# Autodesk Inventor assembly: ARM_039_MiddleRoller
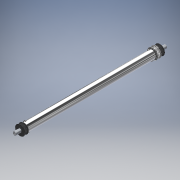
[picture p0: Inventor's stored thumbnail of the model, 180x180]
Saved by Autodesk Inventor 2018.3 (Build 223284000, 284)
## iProperties
Created: 2020-02-08
Part Number: ARM_039_MiddleRoller
Document SubType Name: Assembly
Designer: 22turnmaxw
Author: 22turnmaxw
## Documents named in this file (9)
- C:\Users\22barlalex\Documents\GrabCAD\Infinite Recharge 2020\Build season\ARM_039_MiddleRoller.iam
- C:\Users\22barlalex\Documents\GrabCAD\Infinite Recharge 2020\Build season\ARM_038_MiddleRollerTube.ipt
- C:\Users\22barlalex\Documents\GrabCAD\Infinite Recharge 2020\Build season\ARM_015_VersaRoller_Hub_1_2_Hex_Bore_x_1-1_8_OD_Aluminum_217-5895.ipt
- C:\Users\22barlalex\Documents\GrabCAD\Infinite Recharge 2020\Build season\ARM_034_36Tx9mm3mmPitchPulley.ipt
- C:\Users\22barlalex\Documents\GrabCAD\Infinite Recharge 2020\Build season\ARM_028_ANSI B18.3 - 10-24 UNC - UNC - 0.1875.ipt
- C:\Users\22barlalex\Documents\GrabCAD\Infinite Recharge 2020\Build season\ARM_027_ANSI B18.3 - 5_16-18 UNC - UNC - 0.5.ipt
- C:\Users\22barlalex\Documents\GrabCAD\Infinite Recharge 2020\Build season\ARM_044_SDP_a_6a53-040df0908.ipt
- C:\Users\22barlalex\Documents\GrabCAD\Infinite Recharge 2020\Build season\ARM_017_VersaRoller_1_2_Hex_Hub_Insert_1_2_Hex_Shaft_x_2-1_2_Long_217-5899.ipt
- C:\Users\22barlalex\Documents\GrabCAD\Infinite Recharge 2020\Build season\ARM_056_ActualMiddleRollerRightHexInsert.ipt
## Components (14 placed, 8 different names)
1. ARM_038_MiddleRollerTube:1 — Mate:1, Mate:2, Mate:3, Mate:4, Mate:32, Mate:33, Tangent:1, Mate:34, Tangent:2, Mate:35, Tangent:3, Mate:36, Tangent:4, Mate:72, Mate:91
2. ARM_015_VersaRoller_Hub_1_2_Hex_Bore_x_1-1_8_OD_Aluminum_217-5895:1 — Mate:1, Mate:2, Mate:32, Mate:80, Mate:90
3. ARM_015_VersaRoller_Hub_1_2_Hex_Bore_x_1-1_8_OD_Aluminum_217-5895:2 — Mate:3, Mate:4, Flush:1, Mate:88
4. ARM_034_36Tx9mm3mmPitchPulley:3 — Mate:70, Mate:71, Flush:1, Mate:87, Mate:89
5. Hexagon Socket Button Head Cap Screw - Inch 10 - 24 x 3/16:1 — Mate:33, Tangent:1
6. Hexagon Socket Button Head Cap Screw - Inch 10 - 24 x 3/16:2 — Mate:34, Tangent:2
7. Hexagon Socket Button Head Cap Screw - Inch 10 - 24 x 3/16:3 — Mate:35, Tangent:3
8. Hexagon Socket Button Head Cap Screw - Inch 10 - 24 x 3/16:4 — Mate:36, Tangent:4
9. Hexagon Socket Button Head Cap Screw - Inch 5/16 - 18 x 1/2:2
10. Hexagon Socket Button Head Cap Screw - Inch 5/16 - 18 x 1/2:3 — Mate:85, Mate:86, Mate:87
11. ARM_044_SDP_a_6a53-040df0908:1 — Mate:70, Mate:71, Mate:72, Mate:93
12. ARM_034_36Tx9mm3mmPitchPulley:4 — Mate:80, Mate:92
13. ARM_017_VersaRoller_1_2_Hex_Hub_Insert_1_2_Hex_Shaft_x_2-1_2_Long_217-5899:1 — Mate:85, Mate:86, Mate:88, Mate:89, Mate:93
14. ARM_056_ActualMiddleRollerRightHexInsert:1 — Mate:90, Mate:91, Mate:92
## Relationships (27: Mate 22, Tangent 4, Flush 1)
- Mate:1: ARM_038_MiddleRollerTube:1 ↔ ARM_015_VersaRoller_Hub_1_2_Hex_Bore_x_1-1_8_OD_Aluminum_217-5895:1
- Mate:2: ARM_038_MiddleRollerTube:1 ↔ ARM_015_VersaRoller_Hub_1_2_Hex_Bore_x_1-1_8_OD_Aluminum_217-5895:1
- Mate:3: ARM_038_MiddleRollerTube:1 ↔ ARM_015_VersaRoller_Hub_1_2_Hex_Bore_x_1-1_8_OD_Aluminum_217-5895:2
- Mate:4: ARM_038_MiddleRollerTube:1 ↔ ARM_015_VersaRoller_Hub_1_2_Hex_Bore_x_1-1_8_OD_Aluminum_217-5895:2
- Mate:32: ARM_038_MiddleRollerTube:1 ↔ ARM_015_VersaRoller_Hub_1_2_Hex_Bore_x_1-1_8_OD_Aluminum_217-5895:1
- Mate:33: ARM_038_MiddleRollerTube:1 ↔ Hexagon Socket Button Head Cap Screw - Inch 10 - 24 x 3/16:1
- Tangent:1: ARM_038_MiddleRollerTube:1 ↔ Hexagon Socket Button Head Cap Screw - Inch 10 - 24 x 3/16:1
- Mate:34: ARM_038_MiddleRollerTube:1 ↔ Hexagon Socket Button Head Cap Screw - Inch 10 - 24 x 3/16:2
- Tangent:2: ARM_038_MiddleRollerTube:1 ↔ Hexagon Socket Button Head Cap Screw - Inch 10 - 24 x 3/16:2
- Mate:35: ARM_038_MiddleRollerTube:1 ↔ Hexagon Socket Button Head Cap Screw - Inch 10 - 24 x 3/16:3
- Tangent:3: ARM_038_MiddleRollerTube:1 ↔ Hexagon Socket Button Head Cap Screw - Inch 10 - 24 x 3/16:3
- Mate:36: ARM_038_MiddleRollerTube:1 ↔ Hexagon Socket Button Head Cap Screw - Inch 10 - 24 x 3/16:4
- Tangent:4: ARM_038_MiddleRollerTube:1 ↔ Hexagon Socket Button Head Cap Screw - Inch 10 - 24 x 3/16:4
- Mate:70: ARM_034_36Tx9mm3mmPitchPulley:3 ↔ ARM_044_SDP_a_6a53-040df0908:1
- Mate:71: ARM_034_36Tx9mm3mmPitchPulley:3 ↔ ARM_044_SDP_a_6a53-040df0908:1
- Mate:72: ARM_038_MiddleRollerTube:1 ↔ ARM_044_SDP_a_6a53-040df0908:1
- Mate:80: ARM_015_VersaRoller_Hub_1_2_Hex_Bore_x_1-1_8_OD_Aluminum_217-5895:1 ↔ ARM_034_36Tx9mm3mmPitchPulley:4
- Flush:1: ARM_015_VersaRoller_Hub_1_2_Hex_Bore_x_1-1_8_OD_Aluminum_217-5895:2 ↔ ARM_034_36Tx9mm3mmPitchPulley:3
- Mate:85: Hexagon Socket Button Head Cap Screw - Inch 5/16 - 18 x 1/2:3 ↔ ARM_017_VersaRoller_1_2_Hex_Hub_Insert_1_2_Hex_Shaft_x_2-1_2_Long_217-5899:1
- Mate:86: Hexagon Socket Button Head Cap Screw - Inch 5/16 - 18 x 1/2:3 ↔ ARM_017_VersaRoller_1_2_Hex_Hub_Insert_1_2_Hex_Shaft_x_2-1_2_Long_217-5899:1
- Mate:87: ARM_034_36Tx9mm3mmPitchPulley:3 ↔ Hexagon Socket Button Head Cap Screw - Inch 5/16 - 18 x 1/2:3
- Mate:88: ARM_015_VersaRoller_Hub_1_2_Hex_Bore_x_1-1_8_OD_Aluminum_217-5895:2 ↔ ARM_017_VersaRoller_1_2_Hex_Hub_Insert_1_2_Hex_Shaft_x_2-1_2_Long_217-5899:1
- Mate:89: ARM_034_36Tx9mm3mmPitchPulley:3 ↔ ARM_017_VersaRoller_1_2_Hex_Hub_Insert_1_2_Hex_Shaft_x_2-1_2_Long_217-5899:1
- Mate:90: ARM_015_VersaRoller_Hub_1_2_Hex_Bore_x_1-1_8_OD_Aluminum_217-5895:1 ↔ ARM_056_ActualMiddleRollerRightHexInsert:1
- Mate:91: ARM_038_MiddleRollerTube:1 ↔ ARM_056_ActualMiddleRollerRightHexInsert:1
- Mate:92: ARM_034_36Tx9mm3mmPitchPulley:4 ↔ ARM_056_ActualMiddleRollerRightHexInsert:1
- Mate:93: ARM_044_SDP_a_6a53-040df0908:1 ↔ ARM_017_VersaRoller_1_2_Hex_Hub_Insert_1_2_Hex_Shaft_x_2-1_2_Long_217-5899:1
